# Autodesk Inventor assembly: MIR_HbFinger01ForChild
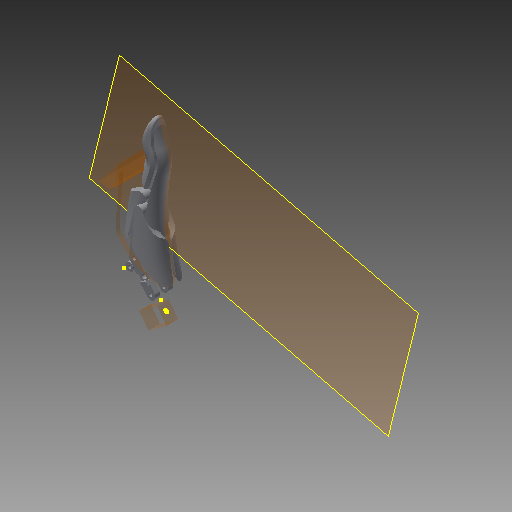
[picture p0: Inventor's stored thumbnail of the model, 512x512]
Saved by Autodesk Inventor 2017 (Build 210142000, 142)
## iProperties
Part Number: MIR_HbFinger01ForChild
Material: 一般
Document SubType Name: Assembly
Designer: sktom
Author: sktom
## Documents named in this file (7)
- D:\OneDrive\CAD\MAJ\hackberry\HACKberry-hardware\3D_69%inlength\Inventor\HbHandForChild\HbFinger01ForChild\MIR_HbFinger01ForChild.iam
- D:\OneDrive\CAD\MAJ\hackberry\HACKberry-hardware\3D_69%inlength\Inventor\HbHandForChild\HbFinger01ForChild\MIR_HbCouplerLinkCover03ForChild.ipt
- D:\OneDrive\CAD\MAJ\hackberry\HACKberry-hardware\3D_69%inlength\Inventor\HbHandForChild\HbFinger01ForChild\MIR_HbCouplerLink02ForChild.ipt
- D:\OneDrive\CAD\MAJ\hackberry\HACKberry-hardware\3D_69%inlength\Inventor\HbHandForChild\HbFinger01ForChild\MIR_HbMiddle-DistalPhalanx02ForChild.ipt
- D:\OneDrive\CAD\MAJ\hackberry\HACKberry-hardware\3D_69%inlength\Inventor\HbHandForChild\HbFinger01ForChild\MIR_HbProximalPhalanx02ForChild.ipt
- D:\OneDrive\CAD\MAJ\hackberry\HACKberry-hardware\3D_69%inlength\Inventor\HbHandForChild\HbFinger01ForChild\MIR_HbProximalPhalanxCover02ForChild.ipt
- D:\OneDrive\CAD\MAJ\hackberry\HACKberry-hardware\3D_69%inlength\Inventor\HbHandForChild\HbFinger01ForChild\MIR_shaft_phi1.5_l6.ipt
## Components (7 placed, 6 different names)
1. MIR_HbCouplerLinkCover03ForChild:1 — 挿入:2, 挿入:1
2. MIR_HbCouplerLink02ForChild:1 — 挿入:2, 挿入:1, 挿入:3, 挿入:8
3. MIR_HbMiddle-DistalPhalanx02ForChild:1 — 挿入:3, 挿入:4, 円柱状:2
4. MIR_HbProximalPhalanx02ForChild:1 — 挿入:6, 挿入:5
5. MIR_HbProximalPhalanxCover02ForChild:1 — 挿入:6, 挿入:5, 挿入:4, 挿入:7
6. MIR_shaft_phi1.5_l6:1 — 挿入:7
7. MIR_shaft_phi1.5_l6:2 — 挿入:8, 円柱状:2
## Relationships (9: Insert 8, CylindricalJoint 1)
- 挿入:2 [Insert]: MIR_HbCouplerLinkCover03ForChild:1 ↔ MIR_HbCouplerLink02ForChild:1
- 挿入:1 [Insert]: MIR_HbCouplerLinkCover03ForChild:1 ↔ MIR_HbCouplerLink02ForChild:1
- 挿入:3 [Insert] (0.4 mm): MIR_HbCouplerLink02ForChild:1 ↔ MIR_HbMiddle-DistalPhalanx02ForChild:1
- 挿入:6 [Insert]: MIR_HbProximalPhalanx02ForChild:1 ↔ MIR_HbProximalPhalanxCover02ForChild:1
- 挿入:5 [Insert]: MIR_HbProximalPhalanx02ForChild:1 ↔ MIR_HbProximalPhalanxCover02ForChild:1
- 挿入:4 [Insert] (0.4 mm): MIR_HbMiddle-DistalPhalanx02ForChild:1 ↔ MIR_HbProximalPhalanxCover02ForChild:1
- 挿入:7 [Insert] (0.5 mm): MIR_HbProximalPhalanxCover02ForChild:1 ↔ MIR_shaft_phi1.5_l6:1
- 挿入:8 [Insert] (0.5 mm): MIR_HbCouplerLink02ForChild:1 ↔ MIR_shaft_phi1.5_l6:2
- 円柱状:2 [CylindricalJoint]: MIR_HbMiddle-DistalPhalanx02ForChild:1 ↔ MIR_shaft_phi1.5_l6:2
